# Autodesk Inventor assembly: SanladererBowdenExtruderMirrored
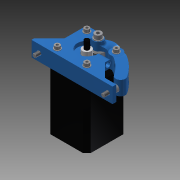
[picture p0: Inventor's stored thumbnail of the model, 180x180]
Saved by Autodesk Inventor 2015 SP1 (Build 190203100, 203)
## iProperties
Created: 2015-01-11
Part Number: SanladererBowdenExtruderMirrored
Document SubType Name: Assembly
Designer: Jack
Mass: 146.796 g
Surface Area: 300.5 cm^2
Volume: 137.998 cm^3
Density: 1.06375 g/cm^3
Author: Jack
Title: Sanlader Extruder Mirrored
## Documents named in this file (11)
- C:\Users\Jack\ownCloud\Projects\CrossBot\InventorModel\Extruder\SanladererBowdenExtruder\SanladererBowdenExtruderMirrored.iam
- C:\Users\Jack\ownCloud\Projects\CrossBot\InventorModel\Extruder\SanladererBowdenExtruder\SanladererBowdenBodyMirrored.ipt
- C:\Users\Jack\ownCloud\Projects\CrossBot\InventorModel\Extruder\SanladererBowdenExtruder\SanladererBowdenArmMirrored.ipt
- C:\Users\Jack\ownCloud\Projects\CrossBot\InventorModel\Electronics\Motors\StepperMotorNema17.ipt
- C:\Users\Jack\ownCloud\Projects\CrossBot\InventorModel\Hardware\Extruder\DriveGearMK8.ipt
- C:\Users\Jack\ownCloud\Projects\CrossBot\InventorModel\Hardware\Bearing\BearingRadialBall\BearingRadialBall624zz.ipt
- C:\Users\Jack\ownCloud\Projects\CrossBot\InventorModel\Hardware\Bolts\SHCS\SHCS3\SHCS3x18.ipt
- C:\Users\Jack\ownCloud\Projects\CrossBot\InventorModel\Hardware\Wahsers\M3Washer.ipt
- C:\Users\Jack\ownCloud\Projects\CrossBot\InventorModel\Hardware\Bolts\SHCS\SHCS4\SHCS4x18.ipt
- C:\Users\Jack\ownCloud\Projects\CrossBot\InventorModel\Hardware\Wahsers\M4Washer.ipt
- C:\Users\Jack\ownCloud\Projects\CrossBot\InventorModel\Hardware\Bolts\SHCS\SHCS4\SHCS4x10.ipt
## Components (19 placed, 10 different names)
1. SanladererBowdenBodyMirrored:1 — Mate:17, Mate:18, Mate:19, Mate:20, Mate:21, Mate:22, Mate:23, Mate:24, Mate:25, Mate:34, Mate:35, Mate:36, Mate:37
2. SanladererBowdenArmMirrored:1 — Mate:26, Mate:27, Mate:29, Mate:30, Mate:31, Mate:32, Mate:33
3. StepperMotorNema17:1 — Mate:17, Mate:18, Mate:19, Mate:30, Mate:31
4. DriveGearMK8:1
5. BearingRadialBall624zz:1 — Mate:28, Mate:29
6. SHCS3x18:1 — Mate:20
7. SHCS3x18:2 — Mate:21
8. SHCS3x18:3 — Mate:32
9. SHCS3x18:4 — Mate:22
10. M3Washer:1 — Mate:25
11. M3Washer:2 — Mate:24
12. M3Washer:3 — Mate:33
13. M3Washer:4 — Mate:23
14. SHCS4x18:1 — Mate:26, Mate:28
15. M4Washer:1 — Mate:27
16. SHCS4x10:1 — Mate:36
17. SHCS4x10:2 — Mate:34
18. M4Washer:2 — Mate:35
19. M4Washer:3 — Mate:37
## Relationships (37: Mate 37)
- [Mate]: StepperMotorNema17:1 ↔ DriveGearMK8:1
- [Mate] (3 mm): StepperMotorNema17:1 ↔ DriveGearMK8:1
- [Mate]: SHCS3x18:4 ↔ M3Washer:4
- [Mate]: SHCS3x18:3 ↔ M3Washer:3
- [Mate]: SHCS3x18:2 ↔ M3Washer:2
- [Mate]: SHCS3x18:1 ↔ M3Washer:1
- [Mate]: SHCS3x18:1 ↔ M3Washer:1
- [Mate]: SHCS3x18:2 ↔ M3Washer:2
- [Mate]: SHCS3x18:3 ↔ M3Washer:3
- [Mate]: SHCS3x18:4 ↔ M3Washer:4
- [Mate]: SHCS4x18:1 ↔ M4Washer:1
- [Mate]: SHCS4x18:1 ↔ M4Washer:1
- [Mate]: SHCS4x10:2 ↔ M4Washer:2
- [Mate]: SHCS4x10:1 ↔ M4Washer:3
- [Mate]: SHCS4x10:1 ↔ M4Washer:3
- [Mate]: SHCS4x10:2 ↔ M4Washer:2
- Mate:17: SanladererBowdenBodyMirrored:1 ↔ StepperMotorNema17:1
- Mate:18: SanladererBowdenBodyMirrored:1 ↔ StepperMotorNema17:1
- Mate:19: SanladererBowdenBodyMirrored:1 ↔ StepperMotorNema17:1
- Mate:20: SanladererBowdenBodyMirrored:1 ↔ SHCS3x18:1
- Mate:21: SanladererBowdenBodyMirrored:1 ↔ SHCS3x18:2
- Mate:22: SanladererBowdenBodyMirrored:1 ↔ SHCS3x18:4
- Mate:23: SanladererBowdenBodyMirrored:1 ↔ M3Washer:4
- Mate:24: SanladererBowdenBodyMirrored:1 ↔ M3Washer:2
- Mate:25: SanladererBowdenBodyMirrored:1 ↔ M3Washer:1
- Mate:26: SanladererBowdenArmMirrored:1 ↔ SHCS4x18:1
- Mate:27: SanladererBowdenArmMirrored:1 ↔ M4Washer:1
- Mate:28: BearingRadialBall624zz:1 ↔ SHCS4x18:1
- Mate:29: SanladererBowdenArmMirrored:1 ↔ BearingRadialBall624zz:1
- Mate:30: SanladererBowdenArmMirrored:1 ↔ StepperMotorNema17:1
- Mate:31: SanladererBowdenArmMirrored:1 ↔ StepperMotorNema17:1
- Mate:32: SanladererBowdenArmMirrored:1 ↔ SHCS3x18:3
- Mate:33: SanladererBowdenArmMirrored:1 ↔ M3Washer:3
- Mate:34: SanladererBowdenBodyMirrored:1 ↔ SHCS4x10:2
- Mate:35: SanladererBowdenBodyMirrored:1 ↔ M4Washer:2
- Mate:36: SanladererBowdenBodyMirrored:1 ↔ SHCS4x10:1
- Mate:37: SanladererBowdenBodyMirrored:1 ↔ M4Washer:3
## Named parameters: d8_d10 = 0 mm, d9_d11 = 3 mm, d10_d15 = 0 mm
